# Autodesk Inventor assembly: Поворотный_модуль_В5
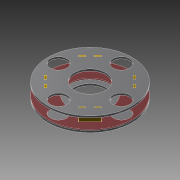
[picture p0: Inventor's stored thumbnail of the model, 180x180]
Saved by Autodesk Inventor 2021.3 (Build 253353000, 353)
## iProperties
Part Number: Поворотный_модуль_В5
Checked By: Якушев
Engr Approved By: Малов
Material: Типовые
Document SubType Name: Assembly
Mfg Approved By: Судаков
Designer: Смирнов
Author: Смирнов
## Documents named in this file (5)
- E:\4. Прочее\1517\Предпрофессиональная олимпиада\Shoter_V5\Поворотный_модуль_В5.iam
- E:\4. Прочее\1517\Предпрофессиональная олимпиада\Shoter_V5\Диск_опорный_В5.ipt
- E:\4. Прочее\1517\Предпрофессиональная олимпиада\Shoter_V5\Диск_базирующий_В5.ipt
- E:\4. Прочее\1517\Предпрофессиональная олимпиада\Shoter_V5\Стойка_В5.ipt
- E:\4. Прочее\1517\Предпрофессиональная олимпиада\Shoter_V5\Диск_верхний_В5.ipt
## Components (7 placed, 4 different names)
1. Диск_опорный_В5:1 — Заподлицо:1, Совмещение:1, Совмещение:2, Совмещение:3
2. Диск_базирующий_В5:1 — Заподлицо:1
3. Диск_верхний_В5:1 — Заподлицо:2
4. Стойка_В5:1 — Совмещение:1, Совмещение:2, Совмещение:3, Заподлицо:2
5. Стойка_В5:2
6. Стойка_В5:3
7. Стойка_В5:4
## Component patterns: (4 elements, first: Стойка_В5:1)
## Relationships (5: Mate 3, Flush 2)
- Заподлицо:1 [Flush]: Диск_опорный_В5:1 ↔ Диск_базирующий_В5:1
- Совмещение:1 [Mate]: Диск_опорный_В5:1 ↔ Стойка_В5:1
- Совмещение:2 [Mate]: Диск_опорный_В5:1 ↔ Стойка_В5:1
- Совмещение:3 [Mate]: Диск_опорный_В5:1 ↔ Стойка_В5:1
- Заподлицо:2 [Flush]: Диск_верхний_В5:1 ↔ Стойка_В5:1
